# Autodesk Inventor assembly: Pressure Vessel, Global Assembly
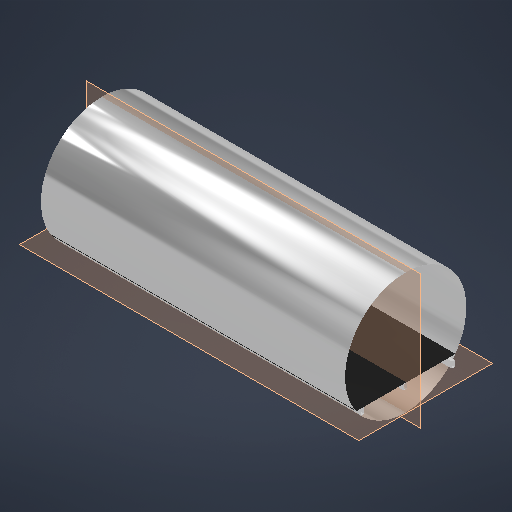
[picture p0: Inventor's stored thumbnail of the model, 512x512]
Saved by Autodesk Inventor 2026 (Build 300175000, 175)
## iProperties
Created: 2025-10-25
Part Number: Pressure Vessel, Global Assembly
Document SubType Name: Assembly
Designer: Brandon Portillo
Author: Brandon Portillo
## Documents named in this file (4)
- C:\Users\anarc\GitHub\TSGC-NASA_Senior_Design\CAD\Pressure Vessel\Pressure Vessel, Global Assembly.iam
- C:\Users\anarc\GitHub\TSGC-NASA_Senior_Design\CAD\Pressure Vessel\Pressure Vessel, Single Part.ipt
- C:\Users\anarc\GitHub\TSGC-NASA_Senior_Design\CAD\Pressure Vessel\Box Beam.ipt
- C:\Users\anarc\GitHub\TSGC-NASA_Senior_Design\CAD\Pressure Vessel\Floor, Uncutt.ipt
## Components (5 placed, 3 different names)
1. Pressure Vessel, Single Part:1 — Flush:1, Flush:2, Tangent:1, Tangent:2, Flush:7, Tangent:3, Tangent:4
2. Box Beam:1 — Flush:2, Flush:3, Flush:6, Mate:1
3. Box Beam:2 — Flush:1, Flush:3, Tangent:1
4. Box Beam:5 — Flush:6, Tangent:2
5. Floor, Uncutt:1 — Mate:1, Flush:7, Tangent:3, Tangent:4, Angle:1
## Relationships (11: Flush 5, Tangent 4, Mate 1, Angle 1)
- Flush:1: Pressure Vessel, Single Part:1 ↔ Box Beam:2
- Flush:2: Pressure Vessel, Single Part:1 ↔ Box Beam:1
- Flush:3: Box Beam:1 ↔ Box Beam:2
- Flush:6: Box Beam:1 ↔ Box Beam:5
- Tangent:1: Pressure Vessel, Single Part:1 ↔ Box Beam:2
- Tangent:2: Pressure Vessel, Single Part:1 ↔ Box Beam:5
- Mate:1: Box Beam:1 ↔ Floor, Uncutt:1
- Flush:7: Pressure Vessel, Single Part:1 ↔ Floor, Uncutt:1
- Tangent:3: Pressure Vessel, Single Part:1 ↔ Floor, Uncutt:1
- Tangent:4: Pressure Vessel, Single Part:1 ↔ Floor, Uncutt:1
- Angle:1 (0 deg): Floor, Uncutt:1
